# Autodesk Inventor assembly: T Bot
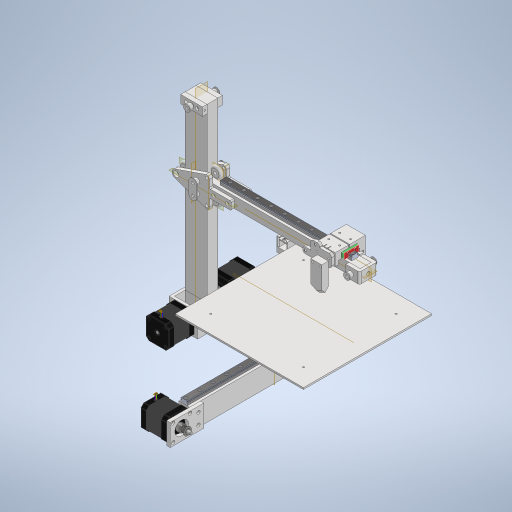
[picture p0: Inventor's stored thumbnail of the model, 512x512]
Saved by Autodesk Inventor 2023.1 (Build 271208000, 208)
## iProperties
Created: 2022-10-29
Part Number: T Bot
Document SubType Name: Assembly
Designer: nicol
Author: nicol
## Documents named in this file (31)
- Y:\Projects\T_Bot_Printer\T Bot.iam
- Y:\Projects\T_Bot_Printer\Cam.ipt
- Y:\Projects\T_Bot_Printer\x 2020.ipt
- Y:\Projects\T_Bot_Printer\XZ Plate.ipt
- Y:\Projects\T_Bot_Printer\Z 2020.ipt
- Y:\Projects\T_Bot_Printer\Wheel.ipt
- Y:\Projects\T_Bot_Printer\MGN-12H\MGN-12H.iam
- Y:\Projects\T_Bot_Printer\Y Base 2040.ipt
- Y:\Projects\T_Bot_Printer\belt pulley.ipt
- Y:\Projects\T_Bot_Printer\NEMA 17.ipt
- Y:\Projects\T_Bot_Printer\GT2 Pulley 16T.ipt
- Y:\Projects\T_Bot_Printer\Print bed.ipt
- Y:\Projects\T_Bot_Printer\build volume.ipt
- Y:\Projects\T_Bot_Printer\Idle Bearing mount2.ipt
- Y:\Projects\T_Bot_Printer\Z Idle belt.ipt
- Y:\Projects\T_Bot_Printer\Y Base 2040 - Copy.ipt
- Y:\Projects\T_Bot_Printer\Motor Mount.ipt
- Y:\Projects\T_Bot_Printer\carriage.ipt
- Y:\Projects\T_Bot_Printer\Belt Holder.ipt
- Y:\Projects\T_Bot_Printer\Belt Retainer Washer.ipt
- Y:\Projects\T_Bot_Printer\hotend.ipt
- Y:\Projects\T_Bot_Printer\electronics mount.ipt
- Y:\Projects\T_Bot_Printer\SKR Mini E3 v3.0.ipt
- Y:\Projects\T_Bot_Printer\Hotend Mount.ipt
- Y:\Projects\T_Bot_Printer\Y Motor Mount.ipt
- Y:\Projects\T_Bot_Printer\Y Center Plate.ipt
- Y:\Projects\T_Bot_Printer\Y Outrigger.ipt
- Y:\Projects\T_Bot_Printer\cf rod.ipt
- Y:\Projects\T_Bot_Printer\Strain Relief.ipt
- Y:\Projects\T_Bot_Printer\Magnet Mount.ipt
- Y:\Projects\T_Bot_Printer\Y Belt.ipt
## Components (59 placed, 30 different names)
1. Cam:1 — Insert:5, Mate:49
2. x 2020:1 — Flush:3, Flush:1, Mate:3, Mate:21, Mate:38, Flush:50, Flush:51, Flush:52, Mate:39, Flush:53, Mate:50, Flush:65, Mate:52, Flush:66
3. XZ Plate:1 — Insert:2, Flush:1, Flush:2, Mate:2, Insert:5, Insert:6, Insert:10, Insert:18, Flush:54
4. Z 2020:1 — Flush:2, Mate:2, Mate:3, Mate:20, Flush:34, Flush:35, Mate:36, Mate:37, Flush:49
5. Wheel:1 — Insert:6, Mate:23
6. Wheel:2 — Insert:2, Flush:3, Mate:22
7. Wheel:3 — Mate:49, Mate:50
8. MGN-12H:1 [sub-assembly] — Mate:20, Flush:34, Flush:35, Insert:31, Insert:32
9. belt pulley:1 — Insert:10, Insert:34
10. belt pulley:2 — Insert:18, Insert:33
11. belt pulley:5 — Insert:24, Insert:44
12. belt pulley:6 — Insert:23, Insert:43
13. NEMA 17:1 — Insert:16
14. NEMA 17:2 — Insert:17, Insert:29, Insert:30
15. GT2 Pulley 16T:1 — Insert:16, Flush:54
16. GT2 Pulley 16T:2 — Insert:17, Flush:55
17. XZ Plate:2 — Mate:21, Mate:22, Mate:23, Flush:55, Insert:35, Insert:36
18. build volume:1
19. Idle Bearing mount2:1 — Mate:36, Mate:37, Flush:49, Insert:23, Insert:24
20. Z Idle belt:1 — Mate:38, Flush:50, Flush:51, Insert:39
21. Z Idle belt:2 — Flush:52, Mate:39, Flush:53, Insert:40
22. MGN-12H:2 [sub-assembly] — Mate:44, Flush:56, Flush:60, Insert:56, Mate:72
23. Y Base 2040:2 — Mate:44, Flush:56, Flush:60, Mate:53, Flush:67, Flush:69, Flush:70, Mate:61, Flush:71, Mate:63, Flush:72, Flush:73, Mate:64
24. Y Base 2040 - Copy:1 — Flush:65, Mate:52, Flush:66, Mate:53, Flush:67, Mate:55, Flush:68, Flush:69, Mate:65, Flush:74
25. Motor Mount:1 — Insert:29, Insert:30, Mate:55, Flush:68
26. carriage:1 — Insert:31, Insert:32, Insert:52, Insert:53
27. Belt Holder:1 — Insert:33, Insert:34
28. Belt Holder:2 — Insert:37, Insert:38
29. belt pulley:7 — Insert:36, Insert:38
30. belt pulley:8 — Insert:35, Insert:37
31. belt pulley:9 — Insert:39, Insert:42
32. belt pulley:10 — Insert:40, Insert:41
33. Belt Retainer Washer:1 — Insert:42
34. Belt Retainer Washer:2 — Insert:41
35. Belt Retainer Washer:3 — Insert:43
36. Belt Retainer Washer:4 — Insert:44
37. hotend:1 — Insert:54, Mate:70
38. NEMA 17:3 — Flush:70, Mate:61, Flush:71, Insert:55, Mate:71
39. GT2 Pulley 16T:3
40. Z Idle belt:3 — Mate:63, Flush:72, Flush:73
41. belt pulley:11
42. Belt Retainer Washer:5
43. electronics mount:1 — Mate:64, Mate:65, Flush:74, Mate:66, Mate:67, Flush:75
44. SKR Mini E3 v3.0:1 — Mate:66, Mate:67, Flush:75
45. Print bed:1 — Insert:61, Mate:82, Insert:62, Angle:5
46. Hotend Mount:1 — Insert:52, Insert:53, Insert:54, Mate:70
47. Y Motor Mount:1 — Insert:55, Mate:71
48. Y Center Plate:1 — Insert:56, Mate:72, Angle:1, Mate:77, Mate:78, Angle:2, Angle:3, Mate:79, Angle:4, Mate:80, Insert:57, Insert:58, Insert:59, Insert:60, Mate:84, Mate:85, Angle:6
49. Y Outrigger:1 — Flush:77, Flush:78, Mate:74, Mate:75, Mate:77, Angle:3
50. Y Outrigger:2 — Flush:78, Mate:75, Angle:2, Mate:79, Mate:81
51. Y Outrigger:3 — Angle:1, Flush:76, Mate:73, Angle:4, Mate:80, Mate:81, Mate:82
52. Y Outrigger:4 — Flush:76, Flush:77, Mate:73, Mate:74, Mate:78, Insert:61
53. cf rod:1 — Insert:57
54. cf rod:2 — Insert:60
55. cf rod:3 — Insert:59
56. cf rod:4 — Insert:58
57. Strain Relief:1 — Insert:62, Angle:5, Flush:79, Mate:83
58. Magnet Mount:1 — Flush:79, Mate:83
59. Y Belt:1 — Mate:84, Mate:85, Angle:6
## Relationships (111: Insert 39, Mate 37, Flush 29, Angle 6)
- Insert:2 (9 mm): XZ Plate:1 ↔ Wheel:2
- Flush:3: x 2020:1 ↔ Wheel:2
- Flush:1: x 2020:1 ↔ XZ Plate:1
- Flush:2: XZ Plate:1 ↔ Z 2020:1
- Mate:2 (2.4 mm): XZ Plate:1 ↔ Z 2020:1
- Insert:5: Cam:1 ↔ XZ Plate:1
- Insert:6 (9 mm): XZ Plate:1 ↔ Wheel:1
- Mate:3 (1 mm): x 2020:1 ↔ Z 2020:1
- Insert:10 (1 mm): XZ Plate:1 ↔ belt pulley:1
- Insert:16: NEMA 17:1 ↔ GT2 Pulley 16T:1
- Insert:17: NEMA 17:2 ↔ GT2 Pulley 16T:2
- Insert:18 (1 mm): XZ Plate:1 ↔ belt pulley:2
- Mate:20: Z 2020:1 ↔ MGN-12H:1
- Flush:34 (20 mm): Z 2020:1 ↔ MGN-12H:1
- Flush:35 (4 mm): Z 2020:1 ↔ MGN-12H:1
- Mate:21 (2.4 mm): x 2020:1 ↔ XZ Plate:2
- Mate:22: Wheel:2 ↔ XZ Plate:2
- Mate:23: Wheel:1 ↔ XZ Plate:2
- Mate:36: Z 2020:1 ↔ Idle Bearing mount2:1
- Mate:37: Z 2020:1 ↔ Idle Bearing mount2:1
- Flush:49: Z 2020:1 ↔ Idle Bearing mount2:1
- Insert:23: belt pulley:6 ↔ Idle Bearing mount2:1
- Insert:24: belt pulley:5 ↔ Idle Bearing mount2:1
- Mate:38: x 2020:1 ↔ Z Idle belt:1
- Flush:50: x 2020:1 ↔ Z Idle belt:1
- Flush:51: x 2020:1 ↔ Z Idle belt:1
- Flush:52: x 2020:1 ↔ Z Idle belt:2
- Mate:39: x 2020:1 ↔ Z Idle belt:2
- Flush:53: x 2020:1 ↔ Z Idle belt:2
- Flush:54: XZ Plate:1 ↔ GT2 Pulley 16T:1
- Flush:55: GT2 Pulley 16T:2 ↔ XZ Plate:2
- Mate:44: MGN-12H:2 ↔ Y Base 2040:2
- Flush:56 (-4 mm): MGN-12H:2 ↔ Y Base 2040:2
- Flush:60: MGN-12H:2 ↔ Y Base 2040:2
- Insert:29: NEMA 17:2 ↔ Motor Mount:1
- Insert:30: NEMA 17:2 ↔ Motor Mount:1
- Insert:31: MGN-12H:1 ↔ carriage:1
- Insert:32: MGN-12H:1 ↔ carriage:1
- Insert:33: belt pulley:2 ↔ Belt Holder:1
- Insert:34: belt pulley:1 ↔ Belt Holder:1
- Insert:35 (1 mm): XZ Plate:2 ↔ belt pulley:8
- Insert:36 (1 mm): XZ Plate:2 ↔ belt pulley:7
- Insert:37: Belt Holder:2 ↔ belt pulley:8
- Insert:38: Belt Holder:2 ↔ belt pulley:7
- Mate:49: Cam:1 ↔ Wheel:3
- Mate:50: x 2020:1 ↔ Wheel:3
- Insert:39: Z Idle belt:1 ↔ belt pulley:9
- Insert:40: Z Idle belt:2 ↔ belt pulley:10
- Insert:41: belt pulley:10 ↔ Belt Retainer Washer:2
- Insert:42: belt pulley:9 ↔ Belt Retainer Washer:1
- Insert:43: belt pulley:6 ↔ Belt Retainer Washer:3
- Insert:44: belt pulley:5 ↔ Belt Retainer Washer:4
- Flush:65: x 2020:1 ↔ Y Base 2040 - Copy:1
- Mate:52: x 2020:1 ↔ Y Base 2040 - Copy:1
- Flush:66: x 2020:1 ↔ Y Base 2040 - Copy:1
- Mate:53: Y Base 2040:2 ↔ Y Base 2040 - Copy:1
- Flush:67: Y Base 2040:2 ↔ Y Base 2040 - Copy:1
- Mate:55: Y Base 2040 - Copy:1 ↔ Motor Mount:1
- Flush:68: Y Base 2040 - Copy:1 ↔ Motor Mount:1
- Flush:69 (-36.75 mm): Y Base 2040:2 ↔ Y Base 2040 - Copy:1
- [Insert]: NEMA 17:3 ↔ GT2 Pulley 16T:3
- Flush:70: Y Base 2040:2 ↔ NEMA 17:3
- Mate:61: Y Base 2040:2 ↔ NEMA 17:3
- Flush:71: Y Base 2040:2 ↔ NEMA 17:3
- [Insert]: Z Idle belt:3 ↔ belt pulley:11
- [Insert]: belt pulley:11 ↔ Belt Retainer Washer:5
- Mate:63: Y Base 2040:2 ↔ Z Idle belt:3
- Flush:72: Y Base 2040:2 ↔ Z Idle belt:3
- Flush:73: Y Base 2040:2 ↔ Z Idle belt:3
- Mate:64: Y Base 2040:2 ↔ electronics mount:1
- Mate:65: Y Base 2040 - Copy:1 ↔ electronics mount:1
- Flush:74: Y Base 2040 - Copy:1 ↔ electronics mount:1
- Mate:66 (6 mm): electronics mount:1 ↔ SKR Mini E3 v3.0:1
- Mate:67 (15 mm): electronics mount:1 ↔ SKR Mini E3 v3.0:1
- Flush:75: electronics mount:1 ↔ SKR Mini E3 v3.0:1
- Insert:52: carriage:1 ↔ Hotend Mount:1
- Insert:53: carriage:1 ↔ Hotend Mount:1
- Insert:54: hotend:1 ↔ Hotend Mount:1
- Mate:70: hotend:1 ↔ Hotend Mount:1
- Insert:55: NEMA 17:3 ↔ Y Motor Mount:1
- Mate:71: NEMA 17:3 ↔ Y Motor Mount:1
- Insert:56: MGN-12H:2 ↔ Y Center Plate:1
- Mate:72: MGN-12H:2 ↔ Y Center Plate:1
- Angle:1 (0 deg): Y Center Plate:1 ↔ Y Outrigger:3
- Flush:76: Y Outrigger:3 ↔ Y Outrigger:4
- Flush:77: Y Outrigger:1 ↔ Y Outrigger:4
- Flush:78: Y Outrigger:1 ↔ Y Outrigger:2
- Mate:73 (170 mm): Y Outrigger:3 ↔ Y Outrigger:4
- Mate:74 (170 mm): Y Outrigger:1 ↔ Y Outrigger:4
- Mate:75 (170 mm): Y Outrigger:1 ↔ Y Outrigger:2
- Mate:77: Y Center Plate:1 ↔ Y Outrigger:1
- Mate:78: Y Center Plate:1 ↔ Y Outrigger:4
- Angle:2 (180 deg): Y Center Plate:1 ↔ Y Outrigger:2
- Angle:3 (180 deg): Y Center Plate:1 ↔ Y Outrigger:1
- Mate:79: Y Center Plate:1 ↔ Y Outrigger:2
- Angle:4 (180 deg): Y Center Plate:1 ↔ Y Outrigger:3
- Mate:80: Y Center Plate:1 ↔ Y Outrigger:3
- Mate:81 (170 mm): Y Outrigger:2 ↔ Y Outrigger:3
- Insert:57: Y Center Plate:1 ↔ cf rod:1
- Insert:58: Y Center Plate:1 ↔ cf rod:4
- Insert:59: Y Center Plate:1 ↔ cf rod:3
- Insert:60: Y Center Plate:1 ↔ cf rod:2
- Insert:61 (12.7 mm): Print bed:1 ↔ Y Outrigger:4
- Mate:82: Print bed:1 ↔ Y Outrigger:3
- Insert:62: Print bed:1 ↔ Strain Relief:1
- Angle:5 (0 deg): Print bed:1 ↔ Strain Relief:1
- Flush:79 (-14.4 mm): Strain Relief:1 ↔ Magnet Mount:1
- Mate:83: Strain Relief:1 ↔ Magnet Mount:1
- Mate:84: Y Center Plate:1 ↔ Y Belt:1
- Mate:85: Y Center Plate:1 ↔ Y Belt:1
- Angle:6 (0 deg): Y Center Plate:1 ↔ Y Belt:1
## Named parameters: d192_d67 = 0 mm, d197_d165 = 0 mm, d198_d168 = 0 mm
